# Autodesk Inventor assembly: encoder_block
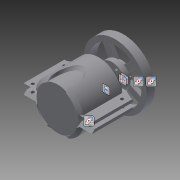
[picture p0: Inventor's stored thumbnail of the model, 180x180]
Saved by Autodesk Inventor 2014 SP1 (Build 180222100, 222)
## iProperties
Created: 2015-07-19
Part Number: encoder_block
Document SubType Name: Assembly
Designer: astralien3000
Author: astralien3000
## Documents named in this file (3)
- C:\Users\astralien3000\Desktop\ceres\meca\v2016\encoder_block.iam
- C:\Users\astralien3000\Desktop\ceres\meca\v2016\encoder.iam
- C:\Users\astralien3000\Desktop\ceres\meca\v2016\encoder_support.ipt
## Components (3 placed, 2 different names)
1. encoder:1 [sub-assembly] — Placage:1, Placage:2, Placage:3, Placage:4, Placage:5, Placage:6
2. encoder_support:1 — Placage:1, Placage:2, Placage:3
3. encoder_support:2 — Placage:4, Placage:5, Placage:6
## Relationships (6: Mate 6)
- Placage:1 [Mate]: encoder:1 ↔ encoder_support:1
- Placage:2 [Mate]: encoder:1 ↔ encoder_support:1
- Placage:3 [Mate]: encoder:1 ↔ encoder_support:1
- Placage:4 [Mate]: encoder:1 ↔ encoder_support:2
- Placage:5 [Mate]: encoder:1 ↔ encoder_support:2
- Placage:6 [Mate]: encoder:1 ↔ encoder_support:2
